# Autodesk Inventor assembly: LD3 Standard
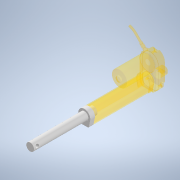
[picture p0: Inventor's stored thumbnail of the model, 180x180]
Saved by Autodesk Inventor 2021 (Build 250183000, 183)
## iProperties
Created: 2014-06-18
Part Number: LD3 Standard
Description: STEP AP203
Document SubType Name: Assembly
Designer: CASE-SMALL2
Sending System: SolidWorks 2012
Preprocessor: SwSTEP 2.0
Title: LD3-100.STEP
Revision Number: ANY
## Documents named in this file (3)
- C:\Users\CASE-SMALL2\Google Drive\Unicorn 2020\CAD_Garbage_Holder\Parts\LD3 Standard.iam
- C:\Users\CASE-SMALL2\Google Drive\Unicorn 2020\CAD_Garbage_Holder\Parts\LD3-Body.ipt
- C:\Users\CASE-SMALL2\Google Drive\Unicorn 2020\CAD_Garbage_Holder\Parts\LD3-Tube.ipt
## Components (2 placed, 2 different names)
1. LD3-Body_1 — Cylindrical:1
2. LD3-Tube_2 — Cylindrical:1
## Relationships (1: CylindricalJoint 1)
- Cylindrical:1: LD3-Body_1 ↔ LD3-Tube_2
